# Autodesk Inventor assembly: robotetz
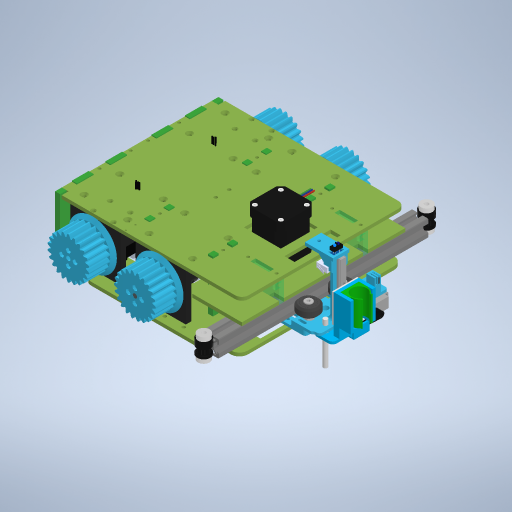
[picture p0: Inventor's stored thumbnail of the model, 512x512]
Saved by Autodesk Inventor 2024.2 (Build 282272000, 272)
## iProperties
Created: 2025-11-16
Part Number: robotetz
Document SubType Name: Assembly
Designer: katya_notebook
Mass: 10483.4 g
Surface Area: 22350.9 cm^2
Volume: 5372.63 cm^3
Density: 1.95127 g/cm^3
Author: katya_notebook
## iProperties of the stored document limit swtch.ipt
Created: 2021-03-18
Part Number: limit swtch
Material: Типовые
Document SubType Name: Modeling
Designer: katya_notebook
Density: 1 g/cm^3
Appearance: По умолчанию
Sending System: SolidWorks 2020
Last Author: medprimetech
Last Saved: 2021-03-18
Author: katya_notebook
## Documents named in this file (37)
- D:\alletz\construction\etz\robotetz.iam
- D:\alletz\construction\полигон\полигон етз.iam
- D:\alletz\construction\мотор левая.iam
- D:\alletz\construction\нижняя пластина.ipt
- D:\alletz\construction\верхняя пластина.ipt
- D:\alletz\construction\маркер.ipt
- D:\alletz\construction\Сервопривод с кареткой.iam
- D:\alletz\construction\TCRT5000\TCRT5000.ipt
- D:\alletz\construction\PROTOBOARD TOP.ipt
- D:\alletz\construction\стенка.ipt
- D:\alletz\construction\стенка 2.ipt
- D:\alletz\construction\Holder 18650 (4 cell)_series_pink\Holder 18650 (4 cell)_series_pink.ipt
- D:\alletz\construction\проставка платы.ipt
- D:\alletz\construction\ступица.ipt
- D:\alletz\construction\колесо\колесо.ipt
- D:\alletz\construction\крышка.ipt
- D:\alletz\construction\колесо\колесо_MIR.ipt
- D:\alletz\construction\ступица_MIR.ipt
- D:\alletz\construction\ручка.ipt
- D:\alletz\construction\TCRT5000\крепление tcrt50002\крепление tcrt50002.ipt
- D:\alletz\construction\красивые провода.ipt
- D:\alletz\construction\etz\robotetz\крепление.ipt
- D:\alletz\construction\Perfil_Aluminio_20x20.ipt
- D:\alletz\construction\муфта.ipt
- D:\alletz\construction\шестерня версия 3.ipt
- D:\alletz\construction\сборка полностью свободной шестерни.iam
- D:\alletz\construction\новая каретка.iam
- D:\alletz\construction\лист.ipt
- D:\alletz\construction\крепление Y.ipt
- D:\alletz\construction\стенка держит стенку.ipt
- D:\alletz\construction\toothed_rack\Nema 17 Stepper.ipt
- D:\alletz\construction\GT2_x_6mm_20_teeht_pulley.ipt
- D:\alletz\construction\washer.ipt
- D:\alletz\construction\крепление шкива боковое.ipt
- D:\alletz\construction\подшипник.ipt
- **D:\alletz\construction\etz\robotetz.iam*LocalDocs*xAaaaqvcaAaaaaaaaAaaaqbwlXb*limit swtch.ipt
- D:\alletz\construction\limit swtch.SLDPRT
## Components (53 placed, 35 different names)
1. полигон етз:1 [sub-assembly] — Заподлицо:8, Заподлицо:53, Заподлицо:83, Заподлицо:84
2. лист:1 — Заподлицо:83, Заподлицо:84
3. крепление:1 — Заподлицо:63, Заподлицо:64
4. ручка:1 — Заподлицо:59, Заподлицо:60, Заподлицо:81
5. стенка 2:1 — Заподлицо:40
6. стенка:1 — Заподлицо:38, Заподлицо:46
7. стенка 2:4 — Совмещение:86, Совмещение:87
8. стенка 2:3 — Совмещение:49
9. стенка 2:2 — Совмещение:84, Совмещение:85, Совмещение:88
10. верхняя пластина:1 — Заподлицо:13, Совмещение:40, Заподлицо:31, Заподлицо:32, Совмещение:47, Заподлицо:47, Заподлицо:48, Заподлицо:49, Совмещение:49, Заподлицо:59, Заподлицо:60, Совмещение:59, Совмещение:60, С поворотом:22, Заподлицо:81, Совмещение:84, Совмещение:85, Совмещение:86, Совмещение:87, Совмещение:88
11. нижняя пластина:1 — Заподлицо:38, Заподлицо:40, Заподлицо:52, Совмещение:56, Совмещение:58, Совмещение:62, Заподлицо:61, Заподлицо:62, Заподлицо:63, Заподлицо:64, С поворотом:13, Заподлицо:71, Заподлицо:72, Заподлицо:73, Совмещение:77, Совмещение:78, Заподлицо:74, Совмещение:79, Заподлицо:75, Заподлицо:76, Заподлицо:78, Совмещение:80, Заподлицо:79, Совмещение:93, Заподлицо:88
12. колесо_MIR:1 — С поворотом:12
13. ступица_MIR:1 — Совмещение:62, Заподлицо:61, Заподлицо:62, С поворотом:12
14. колесо:1 — Совмещение:55, Заподлицо:54
15. крышка:1 — Заподлицо:53, Заподлицо:54
16. ступица:1 — Заподлицо:52, Совмещение:55, Совмещение:56
17. крепление tcrt50002:1 — Совмещение:58, С поворотом:7, Заподлицо:75
18. TCRT5000:1 — С поворотом:7
19. Сервопривод с кареткой:2 [sub-assembly] — С поворотом:13
20. маркер:1 — Совмещение:21, Совмещение:22
21. красивые провода:1 — Совмещение:59
22. красивые провода:2 — Совмещение:60
23. PROTOBOARD TOP:1 — Совмещение:40, Заподлицо:31, Заподлицо:32
24. Holder 18650 (4 cell)_series_pink:1 — Совмещение:47, Заподлицо:46, Заподлицо:47
25. проставка платы:1 — Заподлицо:48, Заподлицо:49, С поворотом:22
26. подшипник:1 — С поворотом:27
27. подшипник:2 — С поворотом:28
28. крепление шкива боковое:2 — Совмещение:99, Заподлицо:93, Совмещение:100
29. подшипник:3 — С поворотом:29
30. подшипник:4 — С поворотом:30
31. GT2_x_6mm_20_teeht_pulley:1 — С поворотом:24, С поворотом:25
32. washer:2 — С поворотом:24
33. стенка держит стенку:3 — Заподлицо:87, Совмещение:91, Совмещение:92
34. limit swtch:1 — Совмещение:103, Совмещение:104
35. новая каретка:1 [sub-assembly] — Совмещение:82, Заподлицо:82, Совмещение:83, Заподлицо:89, Заподлицо:95, Совмещение:101, Совмещение:102, Совмещение:103, Совмещение:104
36. limit swtch:2 — Заподлицо:95, Совмещение:101, Совмещение:102
37. стенка держит стенку:2 — Заподлицо:86, Совмещение:89, Совмещение:90
38. крепление Y:1 — Заподлицо:85, Заподлицо:86, Совмещение:89, Совмещение:90, Заподлицо:87, Совмещение:91, Совмещение:92
39. Nema 17 Stepper:1 — Совмещение:93, С поворотом:25, Совмещение:94, Заподлицо:88
40. Perfil_Aluminio_20x20:1 — Заподлицо:78, Совмещение:80, Заподлицо:79, Совмещение:82, Заподлицо:82, Совмещение:83, Заподлицо:85, Совмещение:94, Заподлицо:89, Заподлицо:90, Совмещение:95, Заподлицо:91, Совмещение:96, Совмещение:97, Совмещение:98, Заподлицо:92, Совмещение:99, Заподлицо:93, Совмещение:100
41. сборка полностью свободной шестерни:1 [sub-assembly] — Заподлицо:73, Совмещение:77, Совмещение:78
42. сборка полностью свободной шестерни:2 [sub-assembly] — Заподлицо:74, Совмещение:79, Заподлицо:76
43. муфта:1 — С поворотом:16, Совмещение:71, С поворотом:21
44. муфта:4 — С поворотом:19, Совмещение:74, С поворотом:20
45. шестерня версия 3:1 — С поворотом:19, Совмещение:74
46. шестерня версия 3:4 — С поворотом:16, Совмещение:71
47. мотор левая:1 [sub-assembly] — С поворотом:20, Заподлицо:72
48. мотор левая:2 [sub-assembly] — Заподлицо:71, С поворотом:21
49. GT2_x_6mm_20_teeht_pulley:3 — С поворотом:26, Совмещение:96, Совмещение:98, С поворотом:29, С поворотом:30
50. washer:3 — С поворотом:26, Заподлицо:91
51. washer:1 — С поворотом:23, Заподлицо:90
52. GT2_x_6mm_20_teeht_pulley:2 — С поворотом:23, Совмещение:95, Совмещение:97, С поворотом:27, С поворотом:28
53. крепление шкива боковое:1 — Заподлицо:92
## Relationships (97: Flush 41, Mate 40, RevoluteJoint 16)
- Заподлицо:8 [Flush] (105 mm): полигон етз:1
- Заподлицо:13 [Flush] (-135 mm): верхняя пластина:1
- Совмещение:21 [Mate]: маркер:1
- Совмещение:22 [Mate]: маркер:1
- Совмещение:40 [Mate]: верхняя пластина:1 ↔ PROTOBOARD TOP:1
- Заподлицо:31 [Flush] (135 mm): верхняя пластина:1 ↔ PROTOBOARD TOP:1
- Заподлицо:32 [Flush] (12 mm): верхняя пластина:1 ↔ PROTOBOARD TOP:1
- Заподлицо:38 [Flush]: стенка:1 ↔ нижняя пластина:1
- Заподлицо:40 [Flush]: стенка 2:1 ↔ нижняя пластина:1
- Совмещение:47 [Mate]: верхняя пластина:1 ↔ Holder 18650 (4 cell)_series_pink:1
- Заподлицо:46 [Flush] (15 mm): стенка:1 ↔ Holder 18650 (4 cell)_series_pink:1
- Заподлицо:47 [Flush] (60 mm): верхняя пластина:1 ↔ Holder 18650 (4 cell)_series_pink:1
- Заподлицо:48 [Flush]: верхняя пластина:1 ↔ проставка платы:1
- Заподлицо:49 [Flush]: верхняя пластина:1 ↔ проставка платы:1
- Совмещение:49 [Mate]: стенка 2:3 ↔ верхняя пластина:1
- Заподлицо:52 [Flush]: нижняя пластина:1 ↔ ступица:1
- Совмещение:55 [Mate]: колесо:1 ↔ ступица:1
- Совмещение:56 [Mate]: нижняя пластина:1 ↔ ступица:1
- Заподлицо:53 [Flush]: полигон етз:1 ↔ крышка:1
- Заподлицо:54 [Flush]: колесо:1 ↔ крышка:1
- Заподлицо:59 [Flush]: ручка:1 ↔ верхняя пластина:1
- Заподлицо:60 [Flush]: ручка:1 ↔ верхняя пластина:1
- Совмещение:58 [Mate]: нижняя пластина:1 ↔ крепление tcrt50002:1
- С поворотом:7 [RevoluteJoint]: крепление tcrt50002:1 ↔ TCRT5000:1
- Совмещение:59 [Mate]: верхняя пластина:1 ↔ красивые провода:1
- Совмещение:60 [Mate]: верхняя пластина:1 ↔ красивые провода:2
- Совмещение:62 [Mate]: нижняя пластина:1 ↔ ступица_MIR:1
- Заподлицо:61 [Flush] (-1.125 mm): нижняя пластина:1 ↔ ступица_MIR:1
- Заподлицо:62 [Flush] (31.309 mm): нижняя пластина:1 ↔ ступица_MIR:1
- С поворотом:12 [RevoluteJoint]: колесо_MIR:1 ↔ ступица_MIR:1
- Заподлицо:63 [Flush]: крепление:1 ↔ нижняя пластина:1
- Заподлицо:64 [Flush]: крепление:1 ↔ нижняя пластина:1
- С поворотом:13 [RevoluteJoint] (-32 mm): нижняя пластина:1 ↔ Сервопривод с кареткой:2
- С поворотом:16 [RevoluteJoint]: муфта:1 ↔ шестерня версия 3:4
- Совмещение:71 [Mate]: муфта:1 ↔ шестерня версия 3:4
- С поворотом:19 [RevoluteJoint]: муфта:4 ↔ шестерня версия 3:1
- Совмещение:74 [Mate]: муфта:4 ↔ шестерня версия 3:1
- С поворотом:20 [RevoluteJoint]: муфта:4 ↔ мотор левая:1
- Заподлицо:71 [Flush] (1.5 mm): нижняя пластина:1 ↔ мотор левая:2
- Заподлицо:72 [Flush] (1.5 mm): нижняя пластина:1 ↔ мотор левая:1
- С поворотом:21 [RevoluteJoint]: муфта:1 ↔ мотор левая:2
- Заподлицо:73 [Flush]: нижняя пластина:1 ↔ сборка полностью свободной шестерни:1
- Совмещение:77 [Mate]: нижняя пластина:1 ↔ сборка полностью свободной шестерни:1
- Совмещение:78 [Mate] (67 mm): нижняя пластина:1 ↔ сборка полностью свободной шестерни:1
- Заподлицо:74 [Flush]: нижняя пластина:1 ↔ сборка полностью свободной шестерни:2
- Совмещение:79 [Mate]: нижняя пластина:1 ↔ сборка полностью свободной шестерни:2
- Заподлицо:75 [Flush]: нижняя пластина:1 ↔ крепление tcrt50002:1
- Заподлицо:76 [Flush] (67 mm): нижняя пластина:1 ↔ сборка полностью свободной шестерни:2
- Заподлицо:78 [Flush] (-27.5 mm): нижняя пластина:1 ↔ Perfil_Aluminio_20x20:1
- Совмещение:80 [Mate] (24 mm): нижняя пластина:1 ↔ Perfil_Aluminio_20x20:1
- Заподлицо:79 [Flush]: нижняя пластина:1 ↔ Perfil_Aluminio_20x20:1
- Совмещение:82 [Mate] (0.9 mm): новая каретка:1 ↔ Perfil_Aluminio_20x20:1
- С поворотом:22 [RevoluteJoint]: верхняя пластина:1 ↔ проставка платы:1
- Заподлицо:81 [Flush] (105 mm): ручка:1 ↔ верхняя пластина:1
- Заподлицо:82 [Flush] (-22.75 mm): новая каретка:1 ↔ Perfil_Aluminio_20x20:1
- Совмещение:83 [Mate] (1 mm): новая каретка:1 ↔ Perfil_Aluminio_20x20:1
- Совмещение:84 [Mate]: стенка 2:2 ↔ верхняя пластина:1
- Совмещение:85 [Mate]: стенка 2:2 ↔ верхняя пластина:1
- Совмещение:86 [Mate]: стенка 2:4 ↔ верхняя пластина:1
- Совмещение:87 [Mate]: стенка 2:4 ↔ верхняя пластина:1
- Совмещение:88 [Mate]: стенка 2:2 ↔ верхняя пластина:1
- Заподлицо:83 [Flush]: полигон етз:1 ↔ лист:1
- Заподлицо:84 [Flush]: полигон етз:1 ↔ лист:1
- Заподлицо:85 [Flush]: крепление Y:1 ↔ Perfil_Aluminio_20x20:1
- Заподлицо:86 [Flush]: стенка держит стенку:2 ↔ крепление Y:1
- Совмещение:89 [Mate]: стенка держит стенку:2 ↔ крепление Y:1
- Совмещение:90 [Mate]: стенка держит стенку:2 ↔ крепление Y:1
- Заподлицо:87 [Flush]: стенка держит стенку:3 ↔ крепление Y:1
- Совмещение:91 [Mate]: стенка держит стенку:3 ↔ крепление Y:1
- Совмещение:92 [Mate]: стенка держит стенку:3 ↔ крепление Y:1
- Совмещение:93 [Mate] (-28 mm): нижняя пластина:1 ↔ Nema 17 Stepper:1
- С поворотом:23 [RevoluteJoint]: washer:1 ↔ GT2_x_6mm_20_teeht_pulley:2
- С поворотом:24 [RevoluteJoint]: GT2_x_6mm_20_teeht_pulley:1 ↔ washer:2
- С поворотом:25 [RevoluteJoint]: GT2_x_6mm_20_teeht_pulley:1 ↔ Nema 17 Stepper:1
- Совмещение:94 [Mate] (10 mm): Nema 17 Stepper:1 ↔ Perfil_Aluminio_20x20:1
- Заподлицо:88 [Flush] (76.5 mm): нижняя пластина:1 ↔ Nema 17 Stepper:1
- Заподлицо:89 [Flush] (-100 mm): новая каретка:1 ↔ Perfil_Aluminio_20x20:1
- С поворотом:26 [RevoluteJoint]: GT2_x_6mm_20_teeht_pulley:3 ↔ washer:3
- Заподлицо:90 [Flush] (3.75 mm): Perfil_Aluminio_20x20:1 ↔ washer:1
- Совмещение:95 [Mate] (8 mm): Perfil_Aluminio_20x20:1 ↔ GT2_x_6mm_20_teeht_pulley:2
- Заподлицо:91 [Flush] (3.75 mm): Perfil_Aluminio_20x20:1 ↔ washer:3
- Совмещение:96 [Mate] (8 mm): Perfil_Aluminio_20x20:1 ↔ GT2_x_6mm_20_teeht_pulley:3
- Совмещение:97 [Mate] (-10 mm): Perfil_Aluminio_20x20:1 ↔ GT2_x_6mm_20_teeht_pulley:2
- Совмещение:98 [Mate] (-10 mm): Perfil_Aluminio_20x20:1 ↔ GT2_x_6mm_20_teeht_pulley:3
- Заподлицо:92 [Flush]: Perfil_Aluminio_20x20:1 ↔ крепление шкива боковое:1
- С поворотом:27 [RevoluteJoint]: подшипник:1 ↔ GT2_x_6mm_20_teeht_pulley:2
- С поворотом:28 [RevoluteJoint]: подшипник:2 ↔ GT2_x_6mm_20_teeht_pulley:2
- Совмещение:99 [Mate]: крепление шкива боковое:2 ↔ Perfil_Aluminio_20x20:1
- Заподлицо:93 [Flush]: крепление шкива боковое:2 ↔ Perfil_Aluminio_20x20:1
- Совмещение:100 [Mate] (-3.993 mm): крепление шкива боковое:2 ↔ Perfil_Aluminio_20x20:1
- С поворотом:29 [RevoluteJoint]: подшипник:3 ↔ GT2_x_6mm_20_teeht_pulley:3
- С поворотом:30 [RevoluteJoint]: подшипник:4 ↔ GT2_x_6mm_20_teeht_pulley:3
- Заподлицо:95 [Flush]: новая каретка:1 ↔ limit swtch:2
- Совмещение:101 [Mate] (6 mm): новая каретка:1 ↔ limit swtch:2
- Совмещение:102 [Mate]: новая каретка:1 ↔ limit swtch:2
- Совмещение:103 [Mate]: limit swtch:1 ↔ новая каретка:1
- Совмещение:104 [Mate] (8 mm): limit swtch:1 ↔ новая каретка:1
## Named parameters: Finish1_Area = 0.713334, Finish1_Depth = 0.03 mm, Finish1_Hardness = 60
note: some values were not read from the file. Shown as the stored number, unit unknown: "Finish1_Area", "Finish1_Hardness".
